# Autodesk Inventor assembly: GM12-N20VA-Motor
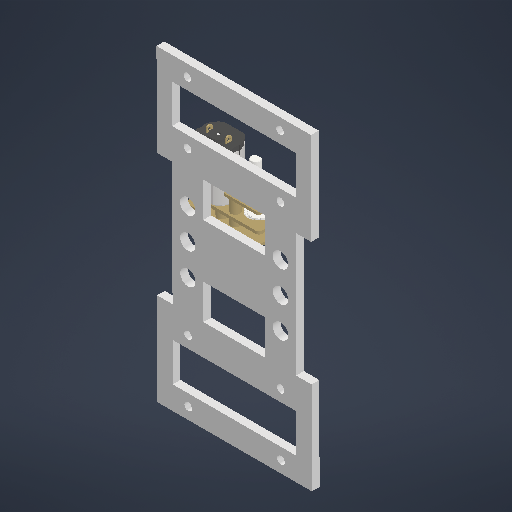
[picture p0: Inventor's stored thumbnail of the model, 512x512]
Saved by Autodesk Inventor 2027 (Build 310192060, 192F)
## iProperties
Created: 1601-01-02
Part Number: GM12-N20VA-Motor
Document SubType Name: Assembly
Designer: loren
Sending System: SOLIDWORKS 2018
Last Saved Date: 2022-07-07
Author: loren
## Documents named in this file (11)
- C:\Users\loren\Desktop\Tesi Magistrale\CAD\FreeBOT\GM12-N20VA-Motor.iam
- C:\Users\loren\Downloads\n20-14.snapshot.1\N20后侧输出轴\GM12-N20VA-Motor\M057-8Y01A.iam
- C:\Users\loren\Downloads\n20-14.snapshot.1\N20后侧输出轴\GM12-N20VA-Motor\减速机支架.ipt
- C:\Users\loren\Downloads\n20-14.snapshot.1\N20后侧输出轴\GM12-N20VA-Motor\十字沉头螺丝.ipt
- C:\Users\loren\Downloads\n20-14.snapshot.1\N20后侧输出轴\GM12-N20VA-Motor\Engrenagem reta21-15.ipt
- C:\Users\loren\Downloads\n20-14.snapshot.1\N20后侧输出轴\GM12-N20VA-Motor\Engrenagem reta27-18.ipt
- C:\Users\loren\Downloads\n20-14.snapshot.1\N20后侧输出轴\GM12-N20VA-Motor\Engrenagem reta28-D.ipt
- C:\Users\loren\Downloads\n20-14.snapshot.1\N20后侧输出轴\GM12-N20VA-Motor\Engrenagem reta25-17.ipt
- C:\Users\loren\Downloads\n20-14.snapshot.1\N20后侧输出轴\GM12-N20VA-Motor\Engrenagem reta12.ipt
- C:\Users\loren\Downloads\n20-14.snapshot.1\N20后侧输出轴\GM12-N20VA-Motor\Engrenagem reta22-11.ipt
- C:\Users\loren\Desktop\Tesi Magistrale\CAD\FreeBOT\chassis.ipt
## Components (12 placed, 12 different names)
1. M057-8Y01A-1 [sub-assembly] — Rigid:1, Rotational:1
2. 减速机支架-1 — Rigid:1, Rigid:2, Rigid:3, Rotational:2, Rotational:3, Rotational:4, Rotational:5, Rotational:6, Rotational:7
3. 十字沉头螺丝-1 — Rigid:3
4. 十字沉头螺丝-2 — Rigid:2
5. Engrenagem reta21-15-1 — Rotational:4
6. Engrenagem reta27-18-1 — Rotational:6
7. Engrenagem reta28-D-1 — Rotational:7
8. Engrenagem reta25-17-1 — Rotational:5
9. Engrenagem reta12-1 — Rotational:1
10. Engrenagem reta22-11-1 — Rotational:2
11. Engrenagem reta21-15-2 — Rotational:3
12. chassis:1
## Relationships (10: RevoluteJoint 7, WeldJoint 3)
- Rigid:1 [WeldJoint]: M057-8Y01A-1 ↔ 减速机支架-1
- Rigid:2 [WeldJoint]: 减速机支架-1 ↔ 十字沉头螺丝-2
- Rigid:3 [WeldJoint]: 减速机支架-1 ↔ 十字沉头螺丝-1
- Rotational:1 [RevoluteJoint]: M057-8Y01A-1 ↔ Engrenagem reta12-1
- Rotational:2 [RevoluteJoint]: 减速机支架-1 ↔ Engrenagem reta22-11-1
- Rotational:3 [RevoluteJoint]: 减速机支架-1 ↔ Engrenagem reta21-15-2
- Rotational:4 [RevoluteJoint]: 减速机支架-1 ↔ Engrenagem reta21-15-1
- Rotational:5 [RevoluteJoint]: 减速机支架-1 ↔ Engrenagem reta25-17-1
- Rotational:6 [RevoluteJoint]: 减速机支架-1 ↔ Engrenagem reta27-18-1
- Rotational:7 [RevoluteJoint]: 减速机支架-1 ↔ Engrenagem reta28-D-1
